# Autodesk Inventor assembly: maquete
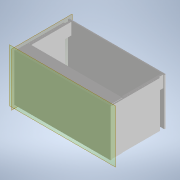
[picture p0: Inventor's stored thumbnail of the model, 180x180]
Saved by Autodesk Inventor 2020 (Build 240168000, 168)
## iProperties
Created: 2021-04-07
Part Number: maquete
Document SubType Name: Assembly
Designer: super
Author: super
## Documents named in this file (6)
- C:\desk\bwmission\maquete\inventor\maquete.iam
- C:\desk\bwmission\maquete\inventor\horizontal.ipt
- C:\desk\bwmission\maquete\inventor\lateralvertical.ipt
- C:\desk\bwmission\maquete\inventor\transversal.ipt
- C:\desk\bwmission\maquete\inventor\vertical apoio.ipt
- C:\desk\bwmission\maquete\inventor\pinho 25x25.ipt
## Components (11 placed, 5 different names)
1. horizontal:1 — Mate:1, Mate:3, Flush:2, Mate:8, Mate:10, Mate:15, Mate:16, Mate:17, Flush:6, Mate:23, Mate:25
2. horizontal:2 — Mate:2, Mate:4, Flush:1, Mate:20, Mate:22
3. lateralvertical:1 — Mate:6, Mate:10, Mate:18, Flush:8, Flush:9, Mate:19, Flush:11, Mate:24
4. lateralvertical:2 — Mate:8, Flush:10, Mate:21, Flush:12, Mate:26
5. pinho 25x25:1 — Mate:15, Flush:8
6. pinho 25x25:3 — Mate:17, Flush:10
7. pinho 25x25:2 — Mate:16, Flush:7, Flush:9
8. transversal:1 — Mate:18, Flush:6, Flush:7, Mate:25, Mate:26
9. vertical apoio:1 — Mate:19, Flush:11, Mate:20
10. vertical apoio:2 — Mate:21, Flush:12, Mate:22
11. transversal:2 — Mate:23, Mate:24
## Relationships (28: Mate 19, Flush 9)
- Mate:1: horizontal:1
- Mate:2 (681 mm): horizontal:2
- Mate:3: horizontal:1
- Mate:4: horizontal:2
- Flush:1: horizontal:2
- Flush:2: horizontal:1
- Mate:6: lateralvertical:1
- Mate:8: horizontal:1 ↔ lateralvertical:2
- Mate:10: horizontal:1 ↔ lateralvertical:1
- Mate:15: horizontal:1 ↔ pinho 25x25:1
- Mate:16: horizontal:1 ↔ pinho 25x25:2
- Mate:17: horizontal:1 ↔ pinho 25x25:3
- Mate:18 (0.5 mm): lateralvertical:1 ↔ transversal:1
- Flush:6: horizontal:1 ↔ transversal:1
- Flush:7: pinho 25x25:2 ↔ transversal:1
- Flush:8 (-309.5 mm): lateralvertical:1 ↔ pinho 25x25:1
- Flush:9 (-606.5 mm): lateralvertical:1 ↔ pinho 25x25:2
- Flush:10 (-309.5 mm): lateralvertical:2 ↔ pinho 25x25:3
- Mate:19: lateralvertical:1 ↔ vertical apoio:1
- Flush:11: lateralvertical:1 ↔ vertical apoio:1
- Mate:20: horizontal:2 ↔ vertical apoio:1
- Mate:21: lateralvertical:2 ↔ vertical apoio:2
- Flush:12: lateralvertical:2 ↔ vertical apoio:2
- Mate:22: horizontal:2 ↔ vertical apoio:2
- Mate:23: horizontal:1 ↔ transversal:2
- Mate:24: lateralvertical:1 ↔ transversal:2
- Mate:25: horizontal:1 ↔ transversal:1
- Mate:26: lateralvertical:2 ↔ transversal:1
